# Autodesk Inventor assembly: 574118 ESBF-BS-100-100-20P---(0)
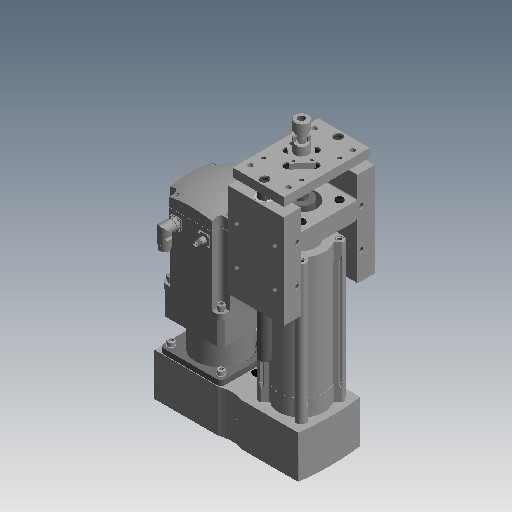
[picture p0: Inventor's stored thumbnail of the model, 512x512]
Saved by Autodesk Inventor 2021 (Build 250183000, 183)
## iProperties
Category: PARTsolutions
Company: FESTO
Part Number: 574118 ESBF-BS-100-100-20P---(0)
Catalog Web Link: www.cadenas.de
Description: ESBF-Electro-cylinder
Vendor: FESTO
Document SubType Name: Assembly
Designer: partserver
Manufacturer: FESTO
Mass: 13053 g
Surface Area: 3910.43 cm^2
Volume: 3059.16 cm^3
Density: 4.26685 g/cm^3
PSOL_IDENT_0: {ATYP=ASSISTANT},{DATA=script=$CADENAS_DATA/23d-libs/festo/webfesto.vbb&M_FAMILY=ESBF&M_GROUP=01&M_P
PSOL_IDENT_1: ARTNO=574118&IDCODE1=ESBF-BS-100-100-20P&IDCODE2=&customer_number_cns=&MATES=1&LOD=HI&LOCKERP=0&SING
PSOL_IDENT_2: LEPART=1}
NB: 574118 ESBF-BS-100-100-20P---(0)
NN: ESBF
NT: Electro-cylinder
NBSYN: $TNR. $TYP.---($HUBST.)
LINA: 574118 ESBF-BS-100-100-20P
CATALOG: Festo
TNR: 574118
TYP: ESBF-BS-100-100-20P
ANT: BS
KDM: 100
HUB: 100
SPI: 20P
HUBST: 0
AM: 40
WH: 51
L1: 33
L2: 324
L3: 39.5
L4: 30
L5: 6.1
L7: 68.5
L8: 5
G: 39
G1: 39
VA: 12
VD: 20
ZJ: 375
KK: M20x1.5
MM: 25
B: 70
D1: 50
D2: 24
D3: 100
BG: 17
EE: G1/8
E: 110
RT: M10
SW1: 22
SW2: 30
SW3: 6
TG: 89
CNSMASSEXACT: 13.053
SUPPLIER: FESTO
ARTICLENO: 574118 ESBF-BS-100-100-20P---(0)
BOMINFO: 574118 ESBF-BS-100-100-20P
CREATOR: CADENAS GmbH
Title: 574118 ESBF-BS-100-100-20P
Author: Cadenas PARTsolutions
Comments: Electro-cylinder
## Documents named in this file (11)
- C:\Users\Santiago Suárez\Documents\GitHub\Dis.-Mecatronico-E6\inventor proyecto\PARTserver0202108060004321756159710e898ce\AIS2021\574118 ESBF-BS-100-100-20P---(0).iam
- C:\Users\Santiago Suárez\Documents\GitHub\Dis.-Mecatronico-E6\inventor proyecto\PARTserver0202108060004321756159710e898ce\AIS2021\ESBF-BS-100-100---(ZR_-_-).ipt
- C:\Users\Santiago Suárez\Documents\GitHub\Dis.-Mecatronico-E6\inventor proyecto\PARTserver0202108060004321756159710e898ce\AIS2021\ESBF-BS-100-100-20P---(KS_0).ipt
- C:\Users\Santiago Suárez\Documents\GitHub\Dis.-Mecatronico-E6\inventor proyecto\PARTserver0202108060004321756159710e898ce\AIS2021\1515746 GUA M28x1_5.ipt
- C:\Users\Santiago Suárez\Documents\GitHub\Dis.-Mecatronico-E6\inventor proyecto\PARTserver0202108060004321756159710e898ce\AIS2021\ESBF-BS-100-ESBF-BS-100---(KSA).ipt
- C:\Users\Santiago Suárez\Documents\GitHub\Dis.-Mecatronico-E6\inventor proyecto\PARTserver0202108060004321756159710e898ce\AIS2021\AIS2021\1725850 EAGF-V2-KF-100-100---(0).iam
- C:\Users\Santiago Suárez\Documents\GitHub\Dis.-Mecatronico-E6\inventor proyecto\PARTserver0202108060004321756159710e898ce\AIS2021\552198 EMGA-120-P-G3-SAS-140.iam
- C:\Users\Santiago Suárez\Documents\GitHub\Dis.-Mecatronico-E6\inventor proyecto\PARTserver0202108060004321756159710e898ce\AIS2021\2803622 EAMM-U-145-D100-120G-188-S1.iam
- C:\Users\Santiago Suárez\Documents\GitHub\Dis.-Mecatronico-E6\inventor proyecto\PARTserver0202108060004321756159710e898ce\1574628 EMMS-AS-140-S-HV-RS.ipt
- C:\Users\Santiago Suárez\Documents\GitHub\Dis.-Mecatronico-E6\inventor proyecto\Cardan\cardan.iam
- C:\Users\Santiago Suárez\Documents\GitHub\Dis.-Mecatronico-E6\inventor proyecto\conector cardan.ipt
## Components (10 placed, 10 different names)
1. ESBF-BS-100-100---(ZR_-_-):1 — KS_XY@1 <-> ANBAU_XY@2, KS_Z@1 <-> ANBAU_Z@2, KS_YZ@1 <-> ANBAU_YZ@2, GUA_XY@1 <-> ANBAU_XY@4, GUA_Z@1 <-> ANBAU_Z@4, GUA_YZ@1 <-> ANBAU_YZ@4, KSA_XY@1 <-> ANBAU_XY@5, KSA_Z@1 <-> ANBAU_Z@5, KSA_YZ@1 <-> ANBAU_YZ@5, Rigid:5
2. ESBF-BS-100-100-20P---(KS_0):1 — KS_XY@1 <-> ANBAU_XY@2, KS_Z@1 <-> ANBAU_Z@2, KS_YZ@1 <-> ANBAU_YZ@2, Rigid:1
3. 1515746 GUA M28x1_5:1 — GUA_XY@1 <-> ANBAU_XY@4, GUA_Z@1 <-> ANBAU_Z@4, GUA_YZ@1 <-> ANBAU_YZ@4
4. ESBF-BS-100-ESBF-BS-100---(KSA):1 — KSA_XY@1 <-> ANBAU_XY@5, KSA_Z@1 <-> ANBAU_Z@5, KSA_YZ@1 <-> ANBAU_YZ@5
5. 1725850 EAGF-V2-KF-100-100---(0):1 [sub-assembly] — Rigid:1, Mate:9, Mate:10
6. 552198 EMGA-120-P-G3-SAS-140:1 [sub-assembly] — Rigid:2, Rigid:3
7. 2803622 EAMM-U-145-D100-120G-188-S1:1 [sub-assembly] — Rigid:3, Rigid:5
8. 1574628 EMMS-AS-140-S-HV-RS:1 — Rigid:2
9. cardan:1 [sub-assembly] — Rigid:4
10. conector cardan:1 — Mate:9, Mate:10, Rigid:4
## Relationships (16: Mate 8, WeldJoint 5, Angle 3)
- KS_XY@1 <-> ANBAU_XY@2 [Mate]: ESBF-BS-100-100---(ZR_-_-):1 ↔ ESBF-BS-100-100-20P---(KS_0):1
- KS_Z@1 <-> ANBAU_Z@2 [Mate]: ESBF-BS-100-100---(ZR_-_-):1 ↔ ESBF-BS-100-100-20P---(KS_0):1
- KS_YZ@1 <-> ANBAU_YZ@2 [Angle] (0 deg): ESBF-BS-100-100---(ZR_-_-):1 ↔ ESBF-BS-100-100-20P---(KS_0):1
- GUA_XY@1 <-> ANBAU_XY@4 [Mate]: ESBF-BS-100-100---(ZR_-_-):1 ↔ 1515746 GUA M28x1_5:1
- GUA_Z@1 <-> ANBAU_Z@4 [Mate]: ESBF-BS-100-100---(ZR_-_-):1 ↔ 1515746 GUA M28x1_5:1
- GUA_YZ@1 <-> ANBAU_YZ@4 [Angle] (0 deg): ESBF-BS-100-100---(ZR_-_-):1 ↔ 1515746 GUA M28x1_5:1
- KSA_XY@1 <-> ANBAU_XY@5 [Mate]: ESBF-BS-100-100---(ZR_-_-):1 ↔ ESBF-BS-100-ESBF-BS-100---(KSA):1
- KSA_Z@1 <-> ANBAU_Z@5 [Mate]: ESBF-BS-100-100---(ZR_-_-):1 ↔ ESBF-BS-100-ESBF-BS-100---(KSA):1
- KSA_YZ@1 <-> ANBAU_YZ@5 [Angle] (0 deg): ESBF-BS-100-100---(ZR_-_-):1 ↔ ESBF-BS-100-ESBF-BS-100---(KSA):1
- Rigid:1 [WeldJoint]: ESBF-BS-100-100-20P---(KS_0):1 ↔ 1725850 EAGF-V2-KF-100-100---(0):1
- Rigid:2 [WeldJoint]: 552198 EMGA-120-P-G3-SAS-140:1 ↔ 1574628 EMMS-AS-140-S-HV-RS:1
- Rigid:3 [WeldJoint]: 552198 EMGA-120-P-G3-SAS-140:1 ↔ 2803622 EAMM-U-145-D100-120G-188-S1:1
- Rigid:5 [WeldJoint]: ESBF-BS-100-100---(ZR_-_-):1 ↔ 2803622 EAMM-U-145-D100-120G-188-S1:1
- Mate:9: 1725850 EAGF-V2-KF-100-100---(0):1 ↔ conector cardan:1
- Mate:10: 1725850 EAGF-V2-KF-100-100---(0):1 ↔ conector cardan:1
- Rigid:4 [WeldJoint]: cardan:1 ↔ conector cardan:1
